# Autodesk Inventor assembly: LegLinksAssembly
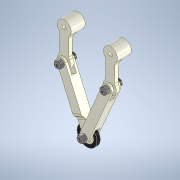
[picture p0: Inventor's stored thumbnail of the model, 180x180]
Saved by Autodesk Inventor 2022 (Build 260153000, 153)
## iProperties
Created: 2021-11-22
Part Number: LegLinksAssembly
Document SubType Name: Assembly
Designer: JK
Mass: 16.0555 g
Surface Area: 94.4419 cm^2
Volume: 9.48605 cm^3
Density: 1.69254 g/cm^3
Author: JK
## Documents named in this file (8)
- C:\Users\JK\Documents\Inventor\N20 Leg Actuator\CADfiles\LegLinksAssembly.iam
- C:\Users\JK\Documents\Inventor\N20 Leg Actuator\CADfiles\LinkA SB.ipt
- C:\Users\JK\Documents\Inventor\N20 Leg Actuator\CADfiles\LinkB SB.ipt
- C:\Users\JK\Documents\Inventor\N20 Leg Actuator\CADfiles\LinkC SB.ipt
- C:\Users\JK\Documents\Inventor\N20 Leg Actuator\CADfiles\Rubberfoot.ipt
- C:\Users\JK\Documents\Inventor\N20 Leg Actuator\CADfiles\M3 Locknut.ipt
- C:\Users\JK\Documents\Inventor\N20 Leg Actuator\CADfiles\683zz.ipt
- C:\Users\JK\Documents\Inventor\N20 Leg Actuator\CADfiles\M3x12SocketBolt.ipt
## Components (14 placed, 7 different names)
1. LinkA SB:1
2. LinkA SB:2
3. LinkB SB:1
4. LinkC SB:1
5. Rubberfoot:1
6. M3 Locknut:1
7. M3 Locknut:2
8. M3 Locknut:3
9. 683zz:1
10. 683zz:2
11. 683zz:3
12. M3x12SocketBolt:1
13. M3x12SocketBolt:2
14. M3x12SocketBolt:3
## Relationships (27: Mate 16, Flush 10, Angle 1)
- [Flush]: LinkA SB:1 ↔ LinkA SB:2
- [Mate]: LinkB SB:1 ↔ LinkC SB:1
- [Flush]: LinkB SB:1 ↔ LinkC SB:1
- [Mate]: LinkC SB:1 ↔ Rubberfoot:1
- [Flush]: M3 Locknut:1 ↔ M3 Locknut:2
- [Flush]: M3 Locknut:2 ↔ M3 Locknut:3
- [Mate]: LinkB SB:1 ↔ M3 Locknut:3
- [Flush]: LinkC SB:1 ↔ Rubberfoot:1
- [Mate]: LinkA SB:1 ↔ 683zz:1
- [Flush]: LinkA SB:1 ↔ 683zz:1
- [Mate]: LinkA SB:2 ↔ 683zz:2
- [Flush]: LinkA SB:2 ↔ 683zz:2
- [Mate] (0.1 mm): LinkB SB:1 ↔ 683zz:1
- [Mate]: LinkA SB:2 ↔ M3x12SocketBolt:1
- [Mate]: LinkC SB:1 ↔ M3x12SocketBolt:3
- [Flush]: M3x12SocketBolt:2 ↔ M3x12SocketBolt:3
- [Mate]: LinkA SB:1 ↔ LinkB SB:1
- [Mate]: LinkA SB:2 ↔ LinkC SB:1
- [Mate]: LinkB SB:1 ↔ M3x12SocketBolt:2
- [Mate]: LinkA SB:1 ↔ M3x12SocketBolt:2
- [Flush]: M3x12SocketBolt:1 ↔ M3x12SocketBolt:2
- [Mate]: M3 Locknut:1 ↔ M3x12SocketBolt:1
- [Mate]: LinkB SB:1 ↔ M3 Locknut:2
- [Mate]: LinkC SB:1 ↔ 683zz:3
- [Flush]: LinkC SB:1 ↔ 683zz:3
- [Mate]: M3 Locknut:3 ↔ M3x12SocketBolt:3
- [Angle] (180 deg): LinkC SB:1 ↔ Rubberfoot:1
